# Autodesk Inventor assembly: AirTank
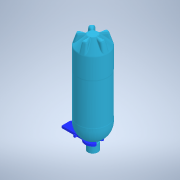
[picture p0: Inventor's stored thumbnail of the model, 180x180]
Saved by Autodesk Inventor 2022.3 (Build 263350000, 350)
## iProperties
Created: 2020-11-12
Part Number: AirTank
Document SubType Name: Assembly
Designer: Hagihara Yuya
Mass: 118.833 g
Surface Area: 1717.25 cm^2
Volume: 34.8334 cm^3
Density: 3.41147 g/cm^3
Author: Hagihara Yuya
## Documents named in this file (4)
- C:\Users\YusukeKunita\Documents\GrabCAD\NHK2022\BasicParts\AirTank(PET-Bottle)\AirTank.iam
- C:\Users\YusukeKunita\Documents\GrabCAD\NHK2022\BasicParts\AirTank(PET-Bottle)\エアタンクペットボトル取付具.ipt
- C:\Users\YusukeKunita\Documents\GrabCAD\NHK2022\BasicParts\AirTank(PET-Bottle)\エアタンクペットボトル抑え２.ipt
- C:\Users\YusukeKunita\Documents\GrabCAD\NHK2022\BasicParts\AirTank(PET-Bottle)\ペットボトル1.5L(ペプシ).ipt
## Components (3 placed, 3 different names)
1. エアタンクペットボトル取付具:1 — 回転:1, 回転:2
2. エアタンクペットボトル抑え２:1 — 回転:1
3. ペットボトル1.5L(ペプシ):1 — 回転:2
## Relationships (2: RevoluteJoint 2)
- 回転:1 [RevoluteJoint]: エアタンクペットボトル取付具:1 ↔ エアタンクペットボトル抑え２:1
- 回転:2 [RevoluteJoint]: エアタンクペットボトル取付具:1 ↔ ペットボトル1.5L(ペプシ):1
